# Autodesk Inventor assembly: LowerJawAssembly
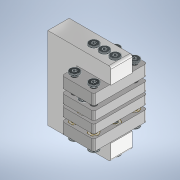
[picture p0: Inventor's stored thumbnail of the model, 180x180]
Saved by Autodesk Inventor 2022 (Build 260153000, 153)
## iProperties
Created: 2021-11-11
Part Number: LowerJawAssembly
Document SubType Name: Assembly
Designer: JK
Author: JK
## Documents named in this file (4)
- C:\Users\JK\Documents\Inventor\UTM\LowerJawAssembly.iam
- C:\Users\JK\Documents\Inventor\UTM\LowerJawLoadCell.ipt
- C:\Users\JK\Documents\Inventor\UTM\ViseAAssembly.iam
- C:\Users\JK\Documents\Inventor\UTM\ViseBAssembly.iam
## Components (5 placed, 3 different names)
1. LowerJawLoadCell:1 — Coincidencia:1, Coincidencia:2, Coincidencia:3, Coincidencia:4, Coincidencia:5, Coincidencia:6
2. ViseAAssembly:1 [sub-assembly] — Coincidencia:1, Coincidencia:2, Coincidencia:3, Coincidencia:7, Nivelación:1
3. ViseAAssembly:2 [sub-assembly] — Coincidencia:4, Coincidencia:5, Coincidencia:6, Coincidencia:8
4. ViseBAssembly:1 [sub-assembly] — Coincidencia:8, Nivelación:2
5. ViseBAssembly:2 [sub-assembly] — Coincidencia:7, Nivelación:1, Nivelación:2
## Relationships (10: Mate 8, Flush 2)
- Coincidencia:1 [Mate]: LowerJawLoadCell:1 ↔ ViseAAssembly:1
- Coincidencia:2 [Mate]: LowerJawLoadCell:1 ↔ ViseAAssembly:1
- Coincidencia:3 [Mate]: LowerJawLoadCell:1 ↔ ViseAAssembly:1
- Coincidencia:4 [Mate]: LowerJawLoadCell:1 ↔ ViseAAssembly:2
- Coincidencia:5 [Mate]: LowerJawLoadCell:1 ↔ ViseAAssembly:2
- Coincidencia:6 [Mate]: LowerJawLoadCell:1 ↔ ViseAAssembly:2
- Coincidencia:7 [Mate]: ViseAAssembly:1 ↔ ViseBAssembly:2
- Nivelación:1 [Flush]: ViseAAssembly:1 ↔ ViseBAssembly:2
- Coincidencia:8 [Mate]: ViseAAssembly:2 ↔ ViseBAssembly:1
- Nivelación:2 [Flush]: ViseBAssembly:1 ↔ ViseBAssembly:2
